# Autodesk Inventor assembly: Rb PEEK
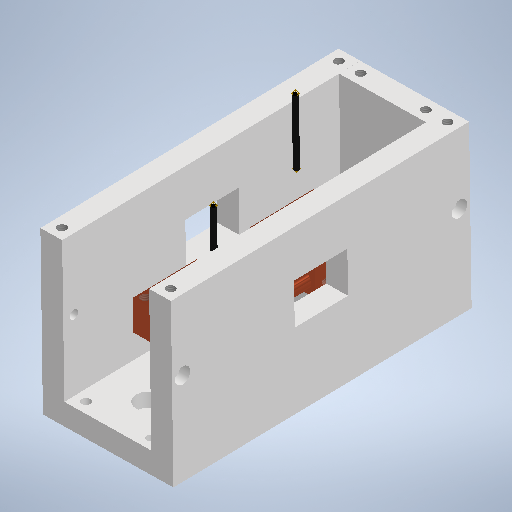
[picture p0: Inventor's stored thumbnail of the model, 512x512]
Saved by Autodesk Inventor 2025.1 (Build 291241000, 241)
## iProperties
Created: 2025-05-09
Part Number: Rb PEEK
Document SubType Name: Assembly
Designer: E. Moreno
Author: E. Moreno
Title: Rb PEEK - Ensamblado
## Documents named in this file (18)
- C:\Users\dell 5810\Documents\M\GitHub\LAFriOC\Rb oven\Rb PEEK\Rb Full.iam
- C:\Users\dell 5810\Documents\M\GitHub\LAFriOC\Rb oven\Rb PEEK\Rb PEEK - Arriba.ipt
- C:\Users\dell 5810\Documents\M\GitHub\LAFriOC\Rb oven\Rb PEEK\Rb PEEK - Largo.ipt
- C:\Users\dell 5810\Documents\M\GitHub\LAFriOC\Rb oven\Rb PEEK\Rb PEEK - Corto con ventana.ipt
- C:\Users\dell 5810\Documents\M\GitHub\LAFriOC\Rb oven\Rb PEEK\Rb PEEK - Soporte.ipt
- C:\Users\dell 5810\Documents\M\GitHub\LAFriOC\Rb oven\Rb PEEK\Rb PEEK - Abajo.ipt
- C:\Users\dell 5810\Documents\M\GitHub\LAFriOC\Rb oven\Rb oven housing\Rb oven housing - Bottom.iam
- E:\Users\USER\Documents\Inventor\Content Center Files\R2025\en-US\AS 1420\AS 1420 - 1973 - M4 x 8.ipt
- C:\Users\dell 5810\Documents\M\GitHub\LAFriOC\Rb oven\Rb parts\Cell.ipt
- C:\Users\dell 5810\Documents\M\GitHub\LAFriOC\Rb oven\Rb oven housing\Rb oven housing - Top.iam
- C:\Users\dell 5810\Documents\M\GitHub\LAFriOC\Rb oven\Rb parts\Heater.ipt
- E:\Users\USER\Documents\Inventor\Content Center Files\R2025\en-US\AS 1420\AS 1420 - 1973 - M4 x 25.ipt
- E:\Users\USER\Documents\Inventor\Content Center Files\R2025\en-US\AS 1420\AS 1420 - 1973 - M4 x 12.ipt
- C:\Users\dell 5810\Documents\M\GitHub\LAFriOC\Rb oven\MS-1L Shield\Shield.iam
- C:\Users\dell 5810\Documents\M\GitHub\LAFriOC\Rb oven\Rb PEEK\Rb Full\AIP\Cable and Harness\Heater Cable1.iam
- C:\Users\dell 5810\Documents\M\GitHub\LAFriOC\Rb oven\Rb PEEK\Rb Full\AIP\Cable and Harness\Heater Cable2.iam
- E:\Users\USER\Documents\Inventor\Content Center Files\R2025\en-US\AS 1420\AS 1420 - 1973 - M6 x 16.ipt
- C:\Users\dell 5810\Documents\M\GitHub\LAFriOC\Rb oven\Rb PEEK\Rb PEEK - Largo_MIR1.ipt
## Components (46 placed, 17 different names)
1. Shield:1 [sub-assembly] — Coincidencia:37
2. Heater Cable1 [sub-assembly]
3. Heater Cable2 [sub-assembly]
4. AS 1420 - Metric M6 x 16:1 — Insert:33
5. AS 1420 - Metric M6 x 16:2 — Insert:34
6. Rb PEEK - Arriba:1 — Coincidencia:1, Coincidencia:2, Coincidencia:3, Coincidencia:5, Coincidencia:6, Coincidencia:33, Insert:9, Insert:10, Insert:11, Insert:12, Insert:13, Insert:14, Insert:15, Insert:16
7. Rb PEEK - Abajo:1 — Coincidencia:21, Coincidencia:22, Coincidencia:23, Coincidencia:29, Coincidencia:30, Coincidencia:34, Insert:21, Insert:24, Insert:25, Insert:26, Insert:27, Insert:28, Insert:29, Insert:30, Insert:31, Insert:32, Insert:33, Insert:34, Coincidencia:37, Coincidencia:38, Coincidencia:39
8. Rb PEEK - Largo:1 — Coincidencia:1, Coincidencia:2, Coincidencia:3, Coincidencia:4, Coincidencia:18, Coincidencia:20, Coincidencia:21, Coincidencia:22, Coincidencia:23, Insert:17, Insert:18
9. Rb PEEK - Largo_MIR1:1 — Coincidencia:38, Coincidencia:39
10. Rb PEEK - Corto con ventana:1 — Coincidencia:4, Coincidencia:5, Coincidencia:6
11. Rb PEEK - Corto con ventana:2 — Coincidencia:18, Coincidencia:20, Coincidencia:33, Coincidencia:34
12. Rb PEEK - Soporte:1 — Coincidencia:29, Insert:1
13. Rb PEEK - Soporte:2 — Coincidencia:30, Coincidencia:31, Insert:2
14. Rb oven housing - Bottom:1 [sub-assembly] — Coincidencia:31, De rotación:1, Insertar:3, Insertar:4
15. Rb oven housing - Top:1 [sub-assembly] — Coincidencia:32, Insert:5, Insert:6, Insert:7, Insert:8
16. Cell:1 — De rotación:1, Coincidencia:32
17. Heater:2 — Insertar:3
18. Heater:3 — Insertar:4
19. AS 1420 - Metric M4 x 8:1 — Insert:1
20. AS 1420 - Metric M4 x 8:2 — Insert:2
21. AS 1420 - Metric M4 x 25:1 — Insert:5
22. AS 1420 - Metric M4 x 25:2 — Insert:6
23. AS 1420 - Metric M4 x 25:3 — Insert:7
24. AS 1420 - Metric M4 x 25:4 — Insert:8
25. AS 1420 - Metric M4 x 25:5 — Insert:9
26. AS 1420 - Metric M4 x 25:6 — Insert:10
27. AS 1420 - Metric M4 x 25:7 — Insert:11
28. AS 1420 - Metric M4 x 25:8 — Insert:12
29. AS 1420 - Metric M4 x 25:9 — Insert:13
30. AS 1420 - Metric M4 x 25:10 — Insert:14
31. AS 1420 - Metric M4 x 25:11 — Insert:15
32. AS 1420 - Metric M4 x 25:12 — Insert:16
33. AS 1420 - Metric M4 x 12:3 — Insert:17
34. AS 1420 - Metric M4 x 12:4 — Insert:18
35. AS 1420 - Metric M4 x 12:5
36. AS 1420 - Metric M4 x 12:6
37. AS 1420 - Metric M4 x 25:13 — Insert:21
38. AS 1420 - Metric M4 x 25:14 — Insert:24
39. AS 1420 - Metric M4 x 25:15 — Insert:25
40. AS 1420 - Metric M4 x 25:16 — Insert:26
41. AS 1420 - Metric M4 x 25:17 — Insert:27
42. AS 1420 - Metric M4 x 25:18 — Insert:28
43. AS 1420 - Metric M4 x 25:19 — Insert:29
44. AS 1420 - Metric M4 x 25:20 — Insert:30
45. AS 1420 - Metric M4 x 12:1 — Insert:31
46. AS 1420 - Metric M4 x 12:2 — Insert:32
## Relationships (51: Insert 30, Mate 20, RevoluteJoint 1)
- Coincidencia:1 [Mate]: Rb PEEK - Arriba:1 ↔ Rb PEEK - Largo:1
- Coincidencia:2 [Mate]: Rb PEEK - Arriba:1 ↔ Rb PEEK - Largo:1
- Coincidencia:3 [Mate]: Rb PEEK - Arriba:1 ↔ Rb PEEK - Largo:1
- Coincidencia:4 [Mate]: Rb PEEK - Largo:1 ↔ Rb PEEK - Corto con ventana:1
- Coincidencia:5 [Mate]: Rb PEEK - Arriba:1 ↔ Rb PEEK - Corto con ventana:1
- Coincidencia:6 [Mate]: Rb PEEK - Arriba:1 ↔ Rb PEEK - Corto con ventana:1
- Coincidencia:18 [Mate]: Rb PEEK - Largo:1 ↔ Rb PEEK - Corto con ventana:2
- Coincidencia:20 [Mate]: Rb PEEK - Largo:1 ↔ Rb PEEK - Corto con ventana:2
- Coincidencia:21 [Mate]: Rb PEEK - Abajo:1 ↔ Rb PEEK - Largo:1
- Coincidencia:22 [Mate]: Rb PEEK - Abajo:1 ↔ Rb PEEK - Largo:1
- Coincidencia:23 [Mate]: Rb PEEK - Abajo:1 ↔ Rb PEEK - Largo:1
- Coincidencia:29 [Mate]: Rb PEEK - Abajo:1 ↔ Rb PEEK - Soporte:1
- Coincidencia:30 [Mate]: Rb PEEK - Abajo:1 ↔ Rb PEEK - Soporte:2
- Coincidencia:31 [Mate]: Rb PEEK - Soporte:2 ↔ Rb oven housing - Bottom:1
- Insert:1: Rb PEEK - Soporte:1 ↔ AS 1420 - Metric M4 x 8:1
- Insert:2: Rb PEEK - Soporte:2 ↔ AS 1420 - Metric M4 x 8:2
- De rotación:1 [RevoluteJoint]: Rb oven housing - Bottom:1 ↔ Cell:1
- Coincidencia:32 [Mate]: Rb oven housing - Top:1 ↔ Cell:1
- Insertar:3 (-10.5 mm): Rb oven housing - Bottom:1 ↔ Heater:2
- Insertar:4 (-10.5 mm): Rb oven housing - Bottom:1 ↔ Heater:3
- Insert:5: Rb oven housing - Top:1 ↔ AS 1420 - Metric M4 x 25:1
- Insert:6: Rb oven housing - Top:1 ↔ AS 1420 - Metric M4 x 25:2
- Insert:7: Rb oven housing - Top:1 ↔ AS 1420 - Metric M4 x 25:3
- Insert:8: Rb oven housing - Top:1 ↔ AS 1420 - Metric M4 x 25:4
- Coincidencia:33 [Mate]: Rb PEEK - Arriba:1 ↔ Rb PEEK - Corto con ventana:2
- Coincidencia:34 [Mate]: Rb PEEK - Abajo:1 ↔ Rb PEEK - Corto con ventana:2
- Insert:9: Rb PEEK - Arriba:1 ↔ AS 1420 - Metric M4 x 25:5
- Insert:10: Rb PEEK - Arriba:1 ↔ AS 1420 - Metric M4 x 25:6
- Insert:11: Rb PEEK - Arriba:1 ↔ AS 1420 - Metric M4 x 25:7
- Insert:12: Rb PEEK - Arriba:1 ↔ AS 1420 - Metric M4 x 25:8
- Insert:13: Rb PEEK - Arriba:1 ↔ AS 1420 - Metric M4 x 25:9
- Insert:14: Rb PEEK - Arriba:1 ↔ AS 1420 - Metric M4 x 25:10
- Insert:15: Rb PEEK - Arriba:1 ↔ AS 1420 - Metric M4 x 25:11
- Insert:16: Rb PEEK - Arriba:1 ↔ AS 1420 - Metric M4 x 25:12
- Insert:17: Rb PEEK - Largo:1 ↔ AS 1420 - Metric M4 x 12:3
- Insert:18: Rb PEEK - Largo:1 ↔ AS 1420 - Metric M4 x 12:4
- Insert:21: Rb PEEK - Abajo:1 ↔ AS 1420 - Metric M4 x 25:13
- Insert:24: Rb PEEK - Abajo:1 ↔ AS 1420 - Metric M4 x 25:14
- Insert:25: Rb PEEK - Abajo:1 ↔ AS 1420 - Metric M4 x 25:15
- Insert:26: Rb PEEK - Abajo:1 ↔ AS 1420 - Metric M4 x 25:16
- Insert:27: Rb PEEK - Abajo:1 ↔ AS 1420 - Metric M4 x 25:17
- Insert:28: Rb PEEK - Abajo:1 ↔ AS 1420 - Metric M4 x 25:18
- Insert:29: Rb PEEK - Abajo:1 ↔ AS 1420 - Metric M4 x 25:19
- Insert:30: Rb PEEK - Abajo:1 ↔ AS 1420 - Metric M4 x 25:20
- Insert:31: Rb PEEK - Abajo:1 ↔ AS 1420 - Metric M4 x 12:1
- Insert:32: Rb PEEK - Abajo:1 ↔ AS 1420 - Metric M4 x 12:2
- Insert:33: AS 1420 - Metric M6 x 16:1 ↔ Rb PEEK - Abajo:1
- Insert:34: AS 1420 - Metric M6 x 16:2 ↔ Rb PEEK - Abajo:1
- Coincidencia:37 [Mate]: Shield:1 ↔ Rb PEEK - Abajo:1
- Coincidencia:38 [Mate]: Rb PEEK - Abajo:1 ↔ Rb PEEK - Largo_MIR1:1
- Coincidencia:39 [Mate]: Rb PEEK - Abajo:1 ↔ Rb PEEK - Largo_MIR1:1
